# Autodesk Inventor assembly: 回路.中身
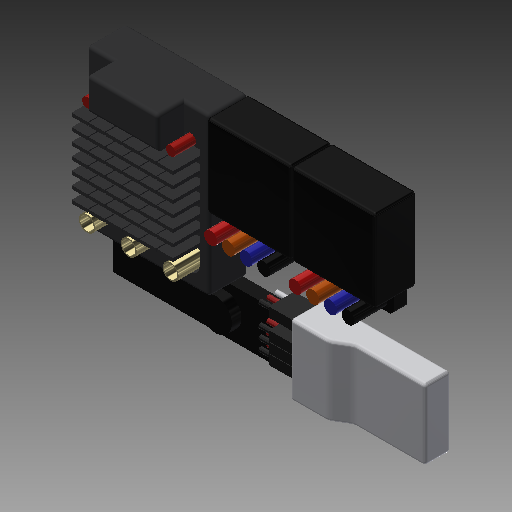
[picture p0: Inventor's stored thumbnail of the model, 512x512]
Saved by Autodesk Inventor 2019 (Build 230136000, 136)
## iProperties
Part Number: 回路.中身
Material: 一般
Document SubType Name: Assembly
Designer: 雪村
Mass: 130.5 g
Surface Area: 248.271 cm^2
Volume: 55.3886 cm^3
Density: 2.35608 g/cm^3
Author: 雪村
## Documents named in this file (5)
- C:\Users\white\Documents\SRDC\SRDC\Inventor_2017\2018年機体\2018年2年機体　雪村\回路.中身.iam
- C:\Users\white\Documents\SRDC\SRDC\Inventor_2017\2018年機体\2018年2年機体　雪村\MC402CR.ipt
- C:\Users\white\Documents\SRDC\SRDC\Inventor_2017\2018年機体\2018年2年機体　雪村\受信機.ipt
- C:\Users\white\Documents\SRDC\SRDC\Inventor_2017\2018年機体\2018年2年機体　雪村\サイドワインダーV3.ipt
- C:\Users\white\Documents\SRDC\SRDC\Inventor_2017\2018年機体\2018年2年機体　雪村\回路.整流器.ipt
## Components (5 placed, 4 different names)
1. MC402CR:1
2. MC402CR:2 — フラッシュ:3, フラッシュ:4, フラッシュ:5
3. 受信機:1 — フラッシュ:5, フラッシュ:7, フラッシュ:8, メイト:4
4. サイドワインダーV3:1 — フラッシュ:3, フラッシュ:4, フラッシュ:6, メイト:3, フラッシュ:9
5. 回路.整流器:1 — フラッシュ:6, フラッシュ:7, メイト:3, フラッシュ:8, フラッシュ:9, メイト:4
## Relationships (13: Flush 9, Mate 4)
- [Mate]: MC402CR:1 ↔ MC402CR:2
- [Flush]: MC402CR:1 ↔ MC402CR:2
- [Flush]: MC402CR:1 ↔ MC402CR:2
- [Mate]: MC402CR:2 ↔ サイドワインダーV3:1
- フラッシュ:3 [Flush]: MC402CR:2 ↔ サイドワインダーV3:1
- フラッシュ:4 [Flush]: MC402CR:2 ↔ サイドワインダーV3:1
- フラッシュ:5 [Flush]: MC402CR:2 ↔ 受信機:1
- フラッシュ:6 [Flush]: サイドワインダーV3:1 ↔ 回路.整流器:1
- フラッシュ:7 [Flush]: 受信機:1 ↔ 回路.整流器:1
- メイト:3 [Mate] (1 mm): サイドワインダーV3:1 ↔ 回路.整流器:1
- フラッシュ:8 [Flush]: 受信機:1 ↔ 回路.整流器:1
- フラッシュ:9 [Flush]: サイドワインダーV3:1 ↔ 回路.整流器:1
- メイト:4 [Mate]: 受信機:1 ↔ 回路.整流器:1
